# Autodesk Inventor assembly: Assembly
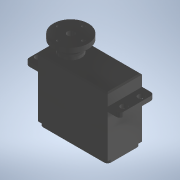
[picture p0: Inventor's stored thumbnail of the model, 180x180]
Saved by Autodesk Inventor 2021 (Build 250183000, 183)
## iProperties
Created: 2020-05-28
Part Number: Assembly
Document SubType Name: Assembly
Designer: izuwa
Author: izuwa
## Documents named in this file (3)
- C:\Users\izuwa\Documents\Inventor\MG996R Servo\Assembly.iam
- C:\Users\izuwa\Documents\Inventor\ironSpidey\BIGSERVO.ipt
- C:\Users\izuwa\Documents\Inventor\ironSpidey\SERVOHORN.ipt
## Components (2 placed, 2 different names)
1. BIGSERVO:1 — Insert:1
2. SERVOHORN:1 — Insert:1
## Relationships (1: Insert 1)
- Insert:1: BIGSERVO:1 ↔ SERVOHORN:1
